# Autodesk Inventor assembly: case_assembly
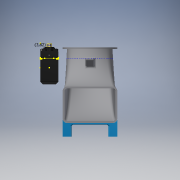
[picture p0: Inventor's stored thumbnail of the model, 180x180]
Saved by Autodesk Inventor 2019 (Build 230136000, 136)
## iProperties
Created: 2019-01-02
Part Number: case_assembly
Document SubType Name: Assembly
Designer: jmc
Author: jmc
## Documents named in this file (18)
- C:\Users\l0086\Desktop\Models\CatFeeder\version2 (fixed enclosure)\version2_newcone.iam
- C:\Users\l0086\Desktop\Models\CatFeeder\Case\version2\case.ipt
- C:\Users\l0086\Desktop\Models\3party\Boards\ArduinoNano\arduino nano.iam
- C:\Users\l0086\Desktop\Models\3party\Boards\Raspberry Pi 3\Raspberry Pi 3.ipt
- C:\Users\l0086\Desktop\Models\3party\Trasformer\Transformer.ipt
- C:\Users\l0086\Desktop\Models\CatFeeder\Case\version2\case_top.ipt
- C:\Users\l0086\Desktop\Models\CatFeeder\Case\version2\case_bottom.ipt
- C:\Users\l0086\Desktop\Models\CatFeeder\Case\version2\Pata.ipt
- C:\Users\l0086\Desktop\Models\CatFeeder\Case\version2\pata_macho.ipt
- C:\Users\l0086\Desktop\Models\CatFeeder\JarCone\version2\cono_nuevo.ipt
- C:\Users\l0086\Desktop\Models\CatFeeder\JarCone\version2\adaptador_cono.ipt
- C:\Users\l0086\Desktop\Models\CatFeeder\Jar\Jar.ipt
- C:\Users\l0086\Desktop\Models\3party\Servos\MG995.ipt
- C:\Users\l0086\Desktop\Models\CatFeeder\Trap\version2\trapdoor_servo.ipt
- C:\Users\l0086\Desktop\Models\CatFeeder\Ramp\version2\ramp.ipt
- C:\Users\l0086\Desktop\Models\CatFeeder\Ramp\version2\ramp_adapter.ipt
- C:\Users\l0086\Desktop\Models\CatFeeder\ServoHolder\version2\servo_holder.ipt
- C:\Users\l0086\Desktop\Models\CatFeeder\Ramp\version2\ramp_holder.ipt
## Components (23 placed, 17 different names)
1. servo_holder:1 — Flush:19
2. case:1
3. case_top:1 — Rigid:15, Rigid:16
4. adaptador_cono:1 — Rotational:6, Rigid:16, Rigid:18
5. case_bottom:1 — Rigid:1, Rigid:3, Rigid:4, Flush:1, Rotational:1, Rigid:6, Rigid:7, Rigid:8, Rigid:15, Flush:12, Flush:17, Flush:18, Mate:1
6. trapdoor_servo:1 — Rotational:6, Rotational:7
7. MG995:1 — Rotational:7, Flush:19, Flush:20
8. Jar:1 — Rigid:17
9. cono_nuevo:1 — Rigid:17, Rigid:18
10. arduino nano:1 [sub-assembly] — Rigid:4
11. Raspberry Pi 3:1 — Rigid:1
12. Transformer:1 — Rigid:3
13. pata_macho:4 — Rotational:5
14. pata_macho:3 — Rotational:3
15. pata_macho:2 — Rotational:4
16. pata_macho:1 — Rotational:2
17. Pata:1 — Flush:1, Rotational:1, Rotational:2
18. Pata:2 — Rigid:8, Rotational:5
19. Pata:3 — Rigid:7, Rotational:3
20. Pata:4 — Rigid:6, Rotational:4
21. ramp_adapter:1 — Flush:17
22. ramp:1 — Flush:12, Flush:18, Mate:1, Flush:20
23. ramp_holder:1
## Relationships (24: WeldJoint 10, RevoluteJoint 7, Flush 6, Mate 1)
- Rigid:1 [WeldJoint]: case_bottom:1 ↔ Raspberry Pi 3:1
- Rigid:3 [WeldJoint]: case_bottom:1 ↔ Transformer:1
- Rigid:4 [WeldJoint]: case_bottom:1 ↔ arduino nano:1
- Flush:1: case_bottom:1 ↔ Pata:1
- Rotational:1 [RevoluteJoint]: case_bottom:1 ↔ Pata:1
- Rigid:6 [WeldJoint]: case_bottom:1 ↔ Pata:4
- Rigid:7 [WeldJoint]: case_bottom:1 ↔ Pata:3
- Rigid:8 [WeldJoint]: case_bottom:1 ↔ Pata:2
- Rotational:2 [RevoluteJoint]: pata_macho:1 ↔ Pata:1
- Rotational:3 [RevoluteJoint]: pata_macho:3 ↔ Pata:3
- Rotational:4 [RevoluteJoint]: pata_macho:2 ↔ Pata:4
- Rotational:5 [RevoluteJoint]: pata_macho:4 ↔ Pata:2
- Rigid:15 [WeldJoint]: case_top:1 ↔ case_bottom:1
- Rotational:6 [RevoluteJoint] (0.4 mm): adaptador_cono:1 ↔ trapdoor_servo:1
- Rotational:7 [RevoluteJoint]: trapdoor_servo:1 ↔ MG995:1
- Flush:12: case_bottom:1 ↔ ramp:1
- Flush:17: case_bottom:1 ↔ ramp_adapter:1
- Rigid:16 [WeldJoint]: case_top:1 ↔ adaptador_cono:1
- Rigid:17 [WeldJoint]: Jar:1 ↔ cono_nuevo:1
- Rigid:18 [WeldJoint]: adaptador_cono:1 ↔ cono_nuevo:1
- Flush:18: case_bottom:1 ↔ ramp:1
- Mate:1: case_bottom:1 ↔ ramp:1
- Flush:19: servo_holder:1 ↔ MG995:1
- Flush:20: MG995:1 ↔ ramp:1
## Named parameters: HOLE_TOLERANCE = 0.15 mm, CASE_TOLERANCE = 0.08 mm
